# Autodesk Inventor assembly: Liu_Inital_Assably
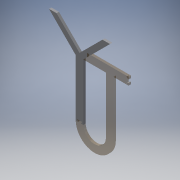
[picture p0: Inventor's stored thumbnail of the model, 180x180]
Saved by Autodesk Inventor 2017 (Build 210142000, 142)
## iProperties
Created: 2016-09-23
Part Number: Liu_Inital_Assably
Document SubType Name: Assembly
Designer: jliu
Author: jliu
## Documents named in this file (3)
- R:\Engineering\Eng16-17\CAD-CAM\Jinyu Liu\Project 2 Initals\Liu_Inital_Assably.iam
- R:\Engineering\Eng16-17\CAD-CAM\Jinyu Liu\Project 2 Initals\Liu_Inital_J.ipt
- R:\Engineering\Eng16-17\CAD-CAM\Jinyu Liu\Project 2 Initals\Liu_Inital_Y.ipt
## Components (2 placed, 2 different names)
1. Liu_Inital_J:1 — Mate:1, Flush:1, Mate:2
2. Liu_Inital_Y:1 — Mate:1, Flush:1, Mate:2
## Relationships (3: Mate 2, Flush 1)
- Mate:1: Liu_Inital_J:1 ↔ Liu_Inital_Y:1
- Flush:1: Liu_Inital_J:1 ↔ Liu_Inital_Y:1
- Mate:2: Liu_Inital_J:1 ↔ Liu_Inital_Y:1
